# Autodesk Inventor assembly: PLA_SetCollar_d6_穴付き
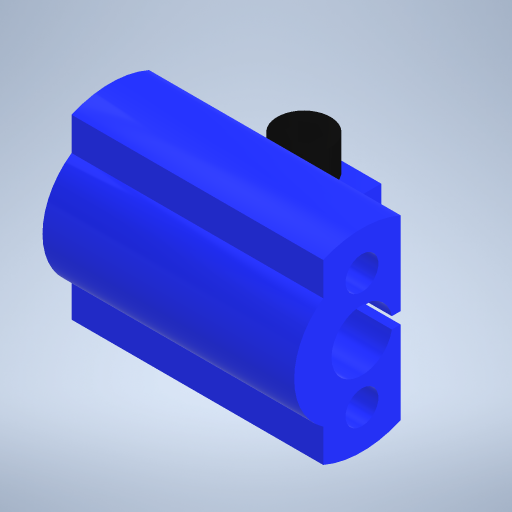
[picture p0: Inventor's stored thumbnail of the model, 512x512]
Saved by Autodesk Inventor 2024 (Build 280153000, 153)
## iProperties
Created: 2020-12-13
Part Number: PLA_SetCollar_d6_穴付き
Document SubType Name: Assembly
Designer: Hagihara Yuya
Author: Hagihara Yuya
## Documents named in this file (4)
- C:\Users\田之上巧太\Documents\Inventor\キャチロボ2024\BasicParts\SetCollar\PLA_SetCollar_d6\PLA_SetCollar_d6_穴付き.iam
- C:\Users\田之上巧太\Documents\Inventor\キャチロボ2024\BasicParts\SetCollar\PLA_SetCollar_d6\Bolt_M3_15_for_SetCollar_d6.ipt
- C:\Users\田之上巧太\Documents\Inventor\キャチロボ2024\BasicParts\SetCollar\PLA_SetCollar_d6\Nut_M3_for_SetCollar.ipt
- C:\Users\田之上巧太\Documents\Inventor\キャチロボ2024\GroundFloor\PLA_SetColor_d6_穴付き copy.ipt
## Components (3 placed, 3 different names)
1. PLA_SetColor_d6_穴付き copy:1 — 回転:1, 回転:2
2. Bolt_M3_15_for_SetCollar_d6:1 — 回転:1
3. Nut_M3_for_SetCollar:1 — 回転:2
## Relationships (2: RevoluteJoint 2)
- 回転:1 [RevoluteJoint]: PLA_SetColor_d6_穴付き copy:1 ↔ Bolt_M3_15_for_SetCollar_d6:1
- 回転:2 [RevoluteJoint]: PLA_SetColor_d6_穴付き copy:1 ↔ Nut_M3_for_SetCollar:1
